# Autodesk Inventor assembly: Pivot Mount
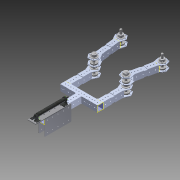
[picture p0: Inventor's stored thumbnail of the model, 180x180]
Saved by Autodesk Inventor 2014 (Build 180170000, 170)
## iProperties
Created: 2014-01-07
Part Number: Pivot Mount
Document SubType Name: Assembly
Designer: Michael
Mass: 1095.79 g
Surface Area: 3529.09 cm^2
Volume: 285.82 cm^3
Density: 3.83384 g/cm^3
Author: Michael
## Documents named in this file (13)
- C:\Users\Michael\Documents\GitHub\2014buildCAD\Funnel Catcher\Pivot Mount.iam
- C:\Users\Michael\Documents\GitHub\2014buildCAD\Funnel Catcher\Vex Pro End Bearing Mount.ipt
- C:\Users\Michael\Documents\GitHub\2014buildCAD\Funnel Catcher\Vex Pro 1x1 rectangular tubing 4 in length.ipt
- C:\Users\Michael\Documents\GitHub\2014buildCAD\Funnel Catcher\3-8 ID 1.125 OD Bearing (6384K348).ipt
- C:\Users\Michael\Documents\GitHub\2014buildCAD\Funnel Catcher\3-8 in ID shaft collar (6435K130).ipt
- C:\Users\Michael\Documents\GitHub\2014buildCAD\Funnel Catcher\Support for Connect Arm to Funnel  (Custom).ipt
- C:\Users\Michael\Documents\GitHub\2014buildCAD\Funnel Catcher\Vex Pro T Gusset.ipt
- C:\Users\Michael\Documents\GitHub\2014buildCAD\Funnel Catcher\Vex Pro 1x1 rectangular tubing 7 in length.ipt
- C:\Users\Michael\Documents\GitHub\2014buildCAD\Funnel Catcher\Vex Pro 90 degree Gusset (Trimmed).ipt
- C:\Users\Michael\Documents\GitHub\2014buildCAD\Funnel Catcher\4 in 3-8 diameter Shaft (6061K419).ipt
- C:\Users\Michael\Documents\GitHub\2014buildCAD\Funnel Catcher\9-16 in Pneumatic Cylinder (3 in Stroke).iam
- C:\Users\Michael\Documents\GitHub\2014buildCAD\Funnel Catcher\Support for 9-16 Piston.ipt
- C:\Users\Michael\Documents\GitHub\2014buildCAD\Funnel Catcher\3 in 3-8 diameter Shaft(6061K418).ipt
## Components (54 placed, 12 different names)
1. Vex Pro End Bearing Mount:1
2. Vex Pro 1x1 rectangular tubing 4 in length:1 — Insert:46, Insert:47
3. Vex Pro End Bearing Mount:2
4. 3-8 ID 1.125 OD Bearing (6384K348):1 — Insert:70
5. 3-8 ID 1.125 OD Bearing (6384K348):2 — Insert:69
6. 3-8 in ID shaft collar (6435K130):1 — Insert:59
7. Vex Pro End Bearing Mount:3
8. Vex Pro 1x1 rectangular tubing 4 in length:2 — Insert:44, Insert:45
9. Vex Pro End Bearing Mount:4
10. 3-8 ID 1.125 OD Bearing (6384K348):3 — Insert:49
11. 3-8 ID 1.125 OD Bearing (6384K348):4 — Insert:50
12. 3-8 in ID shaft collar (6435K130):2 — Insert:50, Insert:55
13. Vex Pro End Bearing Mount:5 — Insert:57, Insert:58
14. Vex Pro End Bearing Mount:6 — Insert:51, Insert:52
15. 3-8 ID 1.125 OD Bearing (6384K348):5 — Insert:59
16. 3-8 ID 1.125 OD Bearing (6384K348):6 — Insert:55
17. 3-8 in ID shaft collar (6435K130):3 — Insert:48, Insert:49
18. Support for Connect Arm to Funnel  (Custom):1 — Insert:79, Insert:80
19. Support for Connect Arm to Funnel  (Custom):2 — Insert:77, Insert:78
20. Vex Pro 1x1 rectangular tubing 4 in length:4 — Insert:51, Insert:52, Insert:57, Insert:58, Insert:87, Insert:88, Insert:93, Insert:94
21. Vex Pro T Gusset:1 — Insert:34, Insert:35, Insert:73, Insert:74
22. Vex Pro T Gusset:2 — Insert:81, Insert:82
23. Vex Pro 1x1 rectangular tubing 7 in length:1 — Insert:34, Insert:35, Insert:36, Insert:37, Insert:38, Insert:39, Insert:40, Insert:41, Insert:42, Insert:43, Insert:81
24. Vex Pro 90 degree Gusset (Trimmed):1 — Insert:36, Insert:37, Insert:46, Insert:47
25. Vex Pro 90 degree Gusset (Trimmed):2 — Insert:38, Insert:39, Insert:44, Insert:45
26. Vex Pro 90 degree Gusset (Trimmed):3 — Insert:42, Insert:43
27. Vex Pro 90 degree Gusset (Trimmed):4 — Insert:40, Insert:41
28. 4 in 3-8 diameter Shaft (6061K419):1 — Insert:66
29. 4 in 3-8 diameter Shaft (6061K419):2 — Insert:48
30. 3-8 in ID shaft collar (6435K130):5 — Insert:66, Insert:67
31. 3-8 in ID shaft collar (6435K130):6 — Insert:68, Insert:69
32. 3-8 in ID shaft collar (6435K130):8 — Insert:70
33. Vex Pro End Bearing Mount:7
34. Vex Pro End Bearing Mount:8
35. 3-8 ID 1.125 OD Bearing (6384K348):7 — Insert:67
36. 3-8 ID 1.125 OD Bearing (6384K348):8 — Insert:68
37. Vex Pro 1x1 rectangular tubing 4 in length:6 — Insert:89, Insert:90, Insert:91, Insert:92
38. 9-16 in Pneumatic Cylinder (3 in Stroke):1 [sub-assembly] — Insert:71, Insert:72
39. Vex Pro 1x1 rectangular tubing 7 in length:2 — Insert:73, Insert:74, Insert:75, Insert:76, Insert:77, Insert:78, Insert:79, Insert:80, Insert:82
40. Support for 9-16 Piston:1 — Insert:71, Insert:72, Insert:75, Insert:76
41. Vex Pro End Bearing Mount:9 — Insert:87, Insert:88
42. 3-8 ID 1.125 OD Bearing (6384K348):9 — Insert:100
43. Vex Pro End Bearing Mount:10 — Insert:89, Insert:90
44. 3-8 ID 1.125 OD Bearing (6384K348):10 — Insert:97
45. Vex Pro End Bearing Mount:11 — Insert:91, Insert:92
46. 3-8 ID 1.125 OD Bearing (6384K348):11 — Insert:96
47. Vex Pro End Bearing Mount:12 — Insert:93, Insert:94
48. 3-8 ID 1.125 OD Bearing (6384K348):12 — Insert:99
49. 3 in 3-8 diameter Shaft(6061K418):1 — Insert:95
50. 3 in 3-8 diameter Shaft(6061K418):2 — Insert:98
51. 3-8 in ID shaft collar (6435K130):9 — Insert:95, Insert:96
52. 3-8 in ID shaft collar (6435K130):10 — Insert:97
53. 3-8 in ID shaft collar (6435K130):11 — Insert:98, Insert:99
54. 3-8 in ID shaft collar (6435K130):12 — Insert:100
## Relationships (78: Insert 78)
- [Insert]: Vex Pro End Bearing Mount:2 ↔ 3-8 ID 1.125 OD Bearing (6384K348):2
- [Insert]: Vex Pro End Bearing Mount:1 ↔ 3-8 ID 1.125 OD Bearing (6384K348):1
- [Insert]: Vex Pro End Bearing Mount:1 ↔ Vex Pro 1x1 rectangular tubing 4 in length:1
- [Insert]: Vex Pro 1x1 rectangular tubing 4 in length:1 ↔ Vex Pro End Bearing Mount:2
- [Insert]: Vex Pro End Bearing Mount:1 ↔ Vex Pro 1x1 rectangular tubing 4 in length:1
- [Insert]: Vex Pro 1x1 rectangular tubing 4 in length:1 ↔ Vex Pro End Bearing Mount:2
- [Insert]: Vex Pro End Bearing Mount:4 ↔ 3-8 ID 1.125 OD Bearing (6384K348):4
- [Insert]: Vex Pro End Bearing Mount:3 ↔ 3-8 ID 1.125 OD Bearing (6384K348):3
- [Insert]: Vex Pro End Bearing Mount:3 ↔ Vex Pro 1x1 rectangular tubing 4 in length:2
- [Insert]: Vex Pro 1x1 rectangular tubing 4 in length:2 ↔ Vex Pro End Bearing Mount:4
- [Insert]: Vex Pro End Bearing Mount:3 ↔ Vex Pro 1x1 rectangular tubing 4 in length:2
- [Insert]: Vex Pro 1x1 rectangular tubing 4 in length:2 ↔ Vex Pro End Bearing Mount:4
- [Insert]: Vex Pro End Bearing Mount:6 ↔ 3-8 ID 1.125 OD Bearing (6384K348):6
- [Insert]: Vex Pro End Bearing Mount:5 ↔ 3-8 ID 1.125 OD Bearing (6384K348):5
- Insert:34: Vex Pro T Gusset:1 ↔ Vex Pro 1x1 rectangular tubing 7 in length:1
- Insert:35: Vex Pro T Gusset:1 ↔ Vex Pro 1x1 rectangular tubing 7 in length:1
- Insert:36: Vex Pro 1x1 rectangular tubing 7 in length:1 ↔ Vex Pro 90 degree Gusset (Trimmed):1
- Insert:37: Vex Pro 1x1 rectangular tubing 7 in length:1 ↔ Vex Pro 90 degree Gusset (Trimmed):1
- Insert:38: Vex Pro 1x1 rectangular tubing 7 in length:1 ↔ Vex Pro 90 degree Gusset (Trimmed):2
- Insert:39: Vex Pro 1x1 rectangular tubing 7 in length:1 ↔ Vex Pro 90 degree Gusset (Trimmed):2
- Insert:40: Vex Pro 1x1 rectangular tubing 7 in length:1 ↔ Vex Pro 90 degree Gusset (Trimmed):4
- Insert:41: Vex Pro 1x1 rectangular tubing 7 in length:1 ↔ Vex Pro 90 degree Gusset (Trimmed):4
- Insert:42: Vex Pro 1x1 rectangular tubing 7 in length:1 ↔ Vex Pro 90 degree Gusset (Trimmed):3
- Insert:43: Vex Pro 1x1 rectangular tubing 7 in length:1 ↔ Vex Pro 90 degree Gusset (Trimmed):3
- Insert:44: Vex Pro 1x1 rectangular tubing 4 in length:2 ↔ Vex Pro 90 degree Gusset (Trimmed):2
- Insert:45: Vex Pro 1x1 rectangular tubing 4 in length:2 ↔ Vex Pro 90 degree Gusset (Trimmed):2
- Insert:46: Vex Pro 1x1 rectangular tubing 4 in length:1 ↔ Vex Pro 90 degree Gusset (Trimmed):1
- Insert:47: Vex Pro 1x1 rectangular tubing 4 in length:1 ↔ Vex Pro 90 degree Gusset (Trimmed):1
- Insert:48 (-1.27 mm): 3-8 in ID shaft collar (6435K130):3 ↔ 4 in 3-8 diameter Shaft (6061K419):2
- Insert:49: 3-8 ID 1.125 OD Bearing (6384K348):3 ↔ 3-8 in ID shaft collar (6435K130):3
- Insert:50: 3-8 ID 1.125 OD Bearing (6384K348):4 ↔ 3-8 in ID shaft collar (6435K130):2
- Insert:51: Vex Pro End Bearing Mount:6 ↔ Vex Pro 1x1 rectangular tubing 4 in length:4
- Insert:52: Vex Pro End Bearing Mount:6 ↔ Vex Pro 1x1 rectangular tubing 4 in length:4
- Insert:55: 3-8 in ID shaft collar (6435K130):2 ↔ 3-8 ID 1.125 OD Bearing (6384K348):6
- Insert:57: Vex Pro End Bearing Mount:5 ↔ Vex Pro 1x1 rectangular tubing 4 in length:4
- Insert:58: Vex Pro End Bearing Mount:5 ↔ Vex Pro 1x1 rectangular tubing 4 in length:4
- Insert:59: 3-8 in ID shaft collar (6435K130):1 ↔ 3-8 ID 1.125 OD Bearing (6384K348):5
- [Insert]: Vex Pro End Bearing Mount:8 ↔ 3-8 ID 1.125 OD Bearing (6384K348):8
- [Insert]: Vex Pro End Bearing Mount:7 ↔ 3-8 ID 1.125 OD Bearing (6384K348):7
- [Insert]: Vex Pro End Bearing Mount:8 ↔ Vex Pro 1x1 rectangular tubing 4 in length:6
- [Insert]: Vex Pro End Bearing Mount:8 ↔ Vex Pro 1x1 rectangular tubing 4 in length:6
- [Insert]: Vex Pro End Bearing Mount:7 ↔ Vex Pro 1x1 rectangular tubing 4 in length:6
- [Insert]: Vex Pro End Bearing Mount:7 ↔ Vex Pro 1x1 rectangular tubing 4 in length:6
- Insert:66: 4 in 3-8 diameter Shaft (6061K419):1 ↔ 3-8 in ID shaft collar (6435K130):5
- Insert:67: 3-8 in ID shaft collar (6435K130):5 ↔ 3-8 ID 1.125 OD Bearing (6384K348):7
- Insert:68: 3-8 in ID shaft collar (6435K130):6 ↔ 3-8 ID 1.125 OD Bearing (6384K348):8
- Insert:69: 3-8 ID 1.125 OD Bearing (6384K348):2 ↔ 3-8 in ID shaft collar (6435K130):6
- Insert:70: 3-8 ID 1.125 OD Bearing (6384K348):1 ↔ 3-8 in ID shaft collar (6435K130):8
- Insert:71: 9-16 in Pneumatic Cylinder (3 in Stroke):1 ↔ Support for 9-16 Piston:1
- Insert:72: 9-16 in Pneumatic Cylinder (3 in Stroke):1 ↔ Support for 9-16 Piston:1
- Insert:73: Vex Pro T Gusset:1 ↔ Vex Pro 1x1 rectangular tubing 7 in length:2
- Insert:74: Vex Pro T Gusset:1 ↔ Vex Pro 1x1 rectangular tubing 7 in length:2
- Insert:75: Vex Pro 1x1 rectangular tubing 7 in length:2 ↔ Support for 9-16 Piston:1
- Insert:76: Vex Pro 1x1 rectangular tubing 7 in length:2 ↔ Support for 9-16 Piston:1
- Insert:77: Support for Connect Arm to Funnel  (Custom):2 ↔ Vex Pro 1x1 rectangular tubing 7 in length:2
- Insert:78: Support for Connect Arm to Funnel  (Custom):2 ↔ Vex Pro 1x1 rectangular tubing 7 in length:2
- Insert:79: Support for Connect Arm to Funnel  (Custom):1 ↔ Vex Pro 1x1 rectangular tubing 7 in length:2
- Insert:80: Support for Connect Arm to Funnel  (Custom):1 ↔ Vex Pro 1x1 rectangular tubing 7 in length:2
- Insert:81: Vex Pro T Gusset:2 ↔ Vex Pro 1x1 rectangular tubing 7 in length:1
- Insert:82: Vex Pro T Gusset:2 ↔ Vex Pro 1x1 rectangular tubing 7 in length:2
- [Insert]: Vex Pro End Bearing Mount:9 ↔ 3-8 ID 1.125 OD Bearing (6384K348):9
- [Insert]: Vex Pro End Bearing Mount:10 ↔ 3-8 ID 1.125 OD Bearing (6384K348):10
- [Insert]: Vex Pro End Bearing Mount:11 ↔ 3-8 ID 1.125 OD Bearing (6384K348):11
- [Insert]: Vex Pro End Bearing Mount:12 ↔ 3-8 ID 1.125 OD Bearing (6384K348):12
- Insert:87: Vex Pro 1x1 rectangular tubing 4 in length:4 ↔ Vex Pro End Bearing Mount:9
- Insert:88: Vex Pro 1x1 rectangular tubing 4 in length:4 ↔ Vex Pro End Bearing Mount:9
- Insert:89: Vex Pro 1x1 rectangular tubing 4 in length:6 ↔ Vex Pro End Bearing Mount:10
- Insert:90: Vex Pro 1x1 rectangular tubing 4 in length:6 ↔ Vex Pro End Bearing Mount:10
- Insert:91: Vex Pro 1x1 rectangular tubing 4 in length:6 ↔ Vex Pro End Bearing Mount:11
- Insert:92: Vex Pro 1x1 rectangular tubing 4 in length:6 ↔ Vex Pro End Bearing Mount:11
- Insert:93: Vex Pro 1x1 rectangular tubing 4 in length:4 ↔ Vex Pro End Bearing Mount:12
- Insert:94: Vex Pro 1x1 rectangular tubing 4 in length:4 ↔ Vex Pro End Bearing Mount:12
- Insert:95: 3 in 3-8 diameter Shaft(6061K418):1 ↔ 3-8 in ID shaft collar (6435K130):9
- Insert:96: 3-8 ID 1.125 OD Bearing (6384K348):11 ↔ 3-8 in ID shaft collar (6435K130):9
- Insert:97: 3-8 ID 1.125 OD Bearing (6384K348):10 ↔ 3-8 in ID shaft collar (6435K130):10
- Insert:98: 3 in 3-8 diameter Shaft(6061K418):2 ↔ 3-8 in ID shaft collar (6435K130):11
- Insert:99: 3-8 ID 1.125 OD Bearing (6384K348):12 ↔ 3-8 in ID shaft collar (6435K130):11
- Insert:100: 3-8 ID 1.125 OD Bearing (6384K348):9 ↔ 3-8 in ID shaft collar (6435K130):12
## Named parameters: d3_d4 = 0 mm, d4_d5 = 0 mm, d8_d30 = 0 mm, d9_d31 = 0 mm, d10_d32 = 0 mm, d11_d3_d4 = 0 mm, d12_d4_d5 = 0 mm, d14_d25 = 0 mm, d18_d3_d4 = 0 mm, d19_d4_d5 = 0 mm, d66_d63 = 0 mm, d67_d64 = 0 mm, d68_d57 = 0 mm, d69_d58 = 0 mm, d70_d18_d3_d4 = 0 mm, d71_d19_d4_d5 = 0 mm, d90_d19_d4_d5 = 0 mm, d91_d19_d4_d5 = 0 mm, d92_d19_d4_d5 = 0 mm, d93_d19_d4_d5 = 0 mm
